# Autodesk Inventor assembly: Rolo_Lap
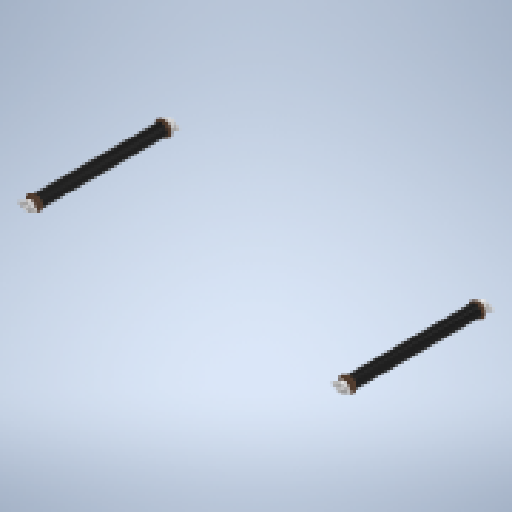
[picture p0: Inventor's stored thumbnail of the model, 512x512]
Saved by Autodesk Inventor 2023 (Build 270158000, 158)
## iProperties
Created: 2025-05-14
Part Number: Rolo_Lap
Document SubType Name: Assembly
Designer: huyqu
Author: huyqu
## Documents named in this file (2)
- E:\TAI LIEU\Final_Project\DONE\BangTai\Rolo_Lap.iam
- E:\TAI LIEU\Final_Project\DONE\BangTai\Rolo.iam
## Components (2 placed, 1 different names)
1. Rolo:1 [sub-assembly] — Flush:1, Mate:1
2. Rolo:2 [sub-assembly] — Flush:1, Mate:1
## Relationships (2: Flush 1, Mate 1)
- Flush:1: Rolo:1 ↔ Rolo:2
- Mate:1 (1950 mm): Rolo:1 ↔ Rolo:2
